# Autodesk Inventor assembly: Test_assembly
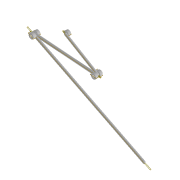
[picture p0: Inventor's stored thumbnail of the model, 180x180]
Saved by Autodesk Inventor 2022 (Build 260153000, 153)
## iProperties
Created: 2022-07-16
Part Number: Test_assembly
Document SubType Name: Assembly
Designer: dell
Author: dell
## Documents named in this file (5)
- D:\xxxx\Uni\Part IV\MECHENG_700\Part_IV_project_CAD\Bird_skeleton_prototypes\Wing_drone_V1\Bird_wing_V2\Test_assembly.iam
- D:\xxxx\Uni\Part IV\MECHENG_700\Part_IV_project_CAD\Bird_skeleton_prototypes\Wing_drone_V1\Bird_wing_V2\Test_gear_p1.ipt
- D:\xxxx\Uni\Part IV\MECHENG_700\Part_IV_project_CAD\Bird_skeleton_prototypes\Wing_drone_V1\Bird_wing_V2\Test_arm_1.ipt
- D:\xxxx\Uni\Part IV\MECHENG_700\Part_IV_project_CAD\Bird_skeleton_prototypes\Wing_drone_V1\Bird_wing_V2\Test_arm_2.ipt
- D:\xxxx\Uni\Part IV\MECHENG_700\Part_IV_project_CAD\Bird_skeleton_prototypes\Wing_drone_V1\Bird_wing_V2\Test_arm_3.ipt
## Components (8 placed, 4 different names)
1. Test_gear_p1:1 — Mate:1, Flush:1, Mate:2, Mate:3, Rotation:2
2. Test_arm_1:1 — Mate:2, Mate:3, Mate:4, Mate:5, Mate:8, Mate:9, Mate:10
3. Test_arm_2:1 — Mate:4, Mate:5, Mate:6, Mate:7, Mate:11, Mate:12, Mate:13, Mate:14, Mate:15, Mate:16
4. Test_arm_3:1 — Mate:6, Mate:7, Mate:17, Mate:18, Mate:19
5. Test_gear_p1:2 — Mate:8, Mate:9, Mate:10, Rotation:1
6. Test_gear_p1:3 — Mate:17, Mate:18, Mate:19, Rotation:1
7. Test_gear_p1:4 — Mate:11, Mate:12, Mate:13, Rotation:2
8. Test_gear_p1:5 — Mate:14, Mate:15, Mate:16
## Relationships (22: Mate 19, RelateRotation 2, Flush 1)
- Mate:1: Test_gear_p1:1
- Flush:1: Test_gear_p1:1
- Mate:2: Test_gear_p1:1 ↔ Test_arm_1:1
- Mate:3: Test_gear_p1:1 ↔ Test_arm_1:1
- Mate:4: Test_arm_1:1 ↔ Test_arm_2:1
- Mate:5: Test_arm_1:1 ↔ Test_arm_2:1
- Mate:6: Test_arm_2:1 ↔ Test_arm_3:1
- Mate:7: Test_arm_2:1 ↔ Test_arm_3:1
- Mate:8: Test_arm_1:1 ↔ Test_gear_p1:2
- Mate:9: Test_arm_1:1 ↔ Test_gear_p1:2
- Mate:10: Test_arm_1:1 ↔ Test_gear_p1:2
- Mate:11: Test_arm_2:1 ↔ Test_gear_p1:4
- Mate:12: Test_arm_2:1 ↔ Test_gear_p1:4
- Mate:13: Test_arm_2:1 ↔ Test_gear_p1:4
- Mate:14: Test_arm_2:1 ↔ Test_gear_p1:5
- Mate:15: Test_arm_2:1 ↔ Test_gear_p1:5
- Mate:16: Test_arm_2:1 ↔ Test_gear_p1:5
- Mate:17: Test_arm_3:1 ↔ Test_gear_p1:3
- Mate:18: Test_arm_3:1 ↔ Test_gear_p1:3
- Mate:19: Test_arm_3:1 ↔ Test_gear_p1:3
- Rotation:1 [RelateRotation] (1 ul): Test_gear_p1:2 ↔ Test_gear_p1:3
- Rotation:2 [RelateRotation] (1 ul): Test_gear_p1:1 ↔ Test_gear_p1:4
